# Autodesk Inventor assembly: Assem1
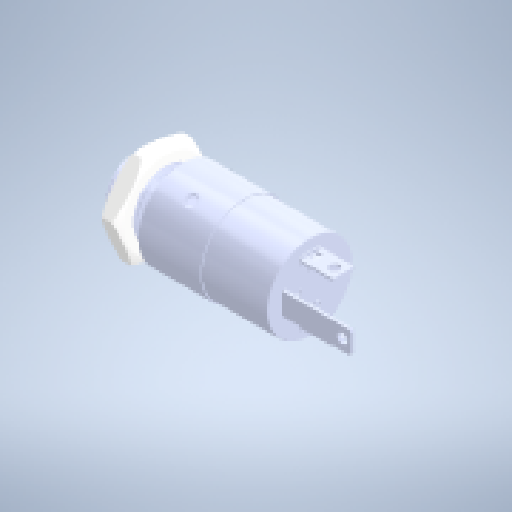
[picture p0: Inventor's stored thumbnail of the model, 512x512]
Saved by Autodesk Inventor 2024 (Build 280153000, 153)
## iProperties
Created: 2015-12-09
Part Number: Assem1
Description: STEP AP214
Document SubType Name: Assembly
Designer: Login
Sending System: SolidWorks 2016
Preprocessor: SwSTEP 2.0
Title: Assem1.STEP
Revision Number: ANY
## Documents named in this file (5)
- D:\Inventor\Repositories\Temperature-Controller\Import\3_5mm_jack.iam
- D:\Inventor\Repositories\Temperature-Controller\Import\front metal.ipt
- D:\Inventor\Repositories\Temperature-Controller\Import\mid plastic.ipt
- D:\Inventor\Repositories\Temperature-Controller\Import\pin.ipt
- D:\Inventor\Repositories\Temperature-Controller\Import\nut_Ä¬ÈÏ¨¨_.ipt
## Components (4 placed, 4 different names)
1. front metal_1 — Insert:1
2. mid plastic_2
3. pin_3
4. nut_Ä¬ÈÏ¨¨__4 — Insert:1
## Relationships (1: Insert 1)
- Insert:1 (1.5 mm): front metal_1 ↔ nut_Ä¬ÈÏ¨¨__4
